# Autodesk Inventor assembly: sensors_haut
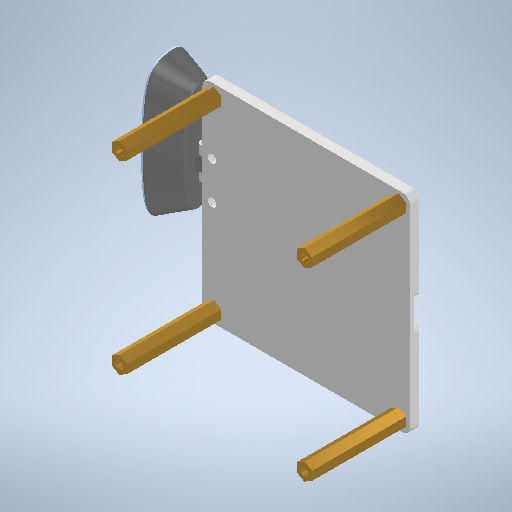
[picture p0: Inventor's stored thumbnail of the model, 512x512]
Saved by Autodesk Inventor 2025.1 (Build 291241000, 241)
## iProperties
Created: 2023-03-21
Part Number: sensors_haut
Document SubType Name: Assembly
Designer: Thomas
Author: Thomas
## Documents named in this file (5)
- C:\Users\baince\Documents\Cours\Ateliers ROB\Autodesk Inventor\Car_Assemblage\Export_Prof\sensors_haut.iam
- C:\Users\baince\Documents\Cours\Ateliers ROB\Autodesk Inventor\Car_2023_Prof_12-10-2023\Workspaces\Espace de travail\support_camera.ipt
- C:\Users\baince\Documents\Cours\Ateliers ROB\Autodesk Inventor\Car_2023_Prof_12-10-2023\Workspaces\Espace de travail\Entretoise-M5-50_806-6651.ipt
- C:\Users\baince\Documents\Cours\Ateliers ROB\Autodesk Inventor\Car_2023_Prof_12-10-2023\Workspaces\Espace de travail\Logitech c270.ipt
- C:\Users\baince\Documents\Cours\Ateliers ROB\Autodesk Inventor\Car_2023_Prof_12-10-2023\Workspaces\Espace de travail\axe_camera.ipt
## Components (7 placed, 4 different names)
1. support_camera:1 — Placage:1, Mate:2, Mate:3, Mate:4, Mate:5, Mate:10, Mate:11, Mate:12
2. Logitech c270:1 — Mate:6, Mate:7, Angle:1
3. axe_camera:1 — Mate:6, Mate:7, Angle:1, Mate:10, Mate:11, Mate:12
4. Entretoise-M5-50_806-6651:1 — Placage:1, Mate:2
5. Entretoise-M5-50_806-6651:2
6. Entretoise-M5-50_806-6651:3
7. Entretoise-M5-50_806-6651:4
## Component patterns: (4 elements, first: Entretoise-M5-50_806-6651:1)
## Relationships (11: Mate 10, Angle 1)
- Placage:1 [Mate]: support_camera:1 ↔ Entretoise-M5-50_806-6651:1
- Mate:2: support_camera:1 ↔ Entretoise-M5-50_806-6651:1
- Mate:3: support_camera:1
- Mate:4: support_camera:1
- Mate:5: support_camera:1
- Mate:6: Logitech c270:1 ↔ axe_camera:1
- Mate:7: Logitech c270:1 ↔ axe_camera:1
- Angle:1 (80 deg): Logitech c270:1 ↔ axe_camera:1
- Mate:10: support_camera:1 ↔ axe_camera:1
- Mate:11: support_camera:1 ↔ axe_camera:1
- Mate:12: support_camera:1 ↔ axe_camera:1
